# Autodesk Inventor assembly: Pok Mk2
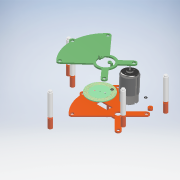
[picture p0: Inventor's stored thumbnail of the model, 180x180]
Saved by Autodesk Inventor 2018.2 (Build 222227000, 227)
## iProperties
Created: 2018-02-07
Part Number: Pok Mk2
Document SubType Name: Assembly
Designer: Moochster
Author: Moochster
## Documents named in this file (10)
- C:\Users\Moochster\OneDrive\Documents\2018 UBC\ELEC 391\Controller\CAD\Pok Mk2.iam
- C:\Users\Moochster\OneDrive\Documents\2018 UBC\ELEC 391\Controller\CAD\JD5B-2655W-R.ipt
- C:\Users\Moochster\OneDrive\Documents\2018 UBC\ELEC 391\Controller\CAD\Encoder Wheel (G16).ipt
- C:\Users\Moochster\OneDrive\Documents\2018 UBC\ELEC 391\Controller\CAD\Pok Yaw Motor Face Mount.ipt
- C:\Users\Moochster\OneDrive\Documents\2018 UBC\ELEC 391\Controller\CAD\Pok Washer I2mmO5mm.ipt
- C:\Users\Moochster\OneDrive\Documents\2018 UBC\ELEC 391\Controller\CAD\Shaft Washer.ipt
- C:\Users\Moochster\OneDrive\Documents\2018 UBC\ELEC 391\Controller\CAD\GP1A52HRJ00F (Large slot detector).ipt
- C:\Users\Moochster\OneDrive\Documents\2018 UBC\ELEC 391\Controller\CAD\Pok X-Carriage Bottom Support.ipt
- C:\Users\Moochster\OneDrive\Documents\2018 UBC\ELEC 391\Controller\CAD\Pok X-Carriage Top Support.ipt
- C:\Users\Moochster\OneDrive\Documents\2018 UBC\ELEC 391\Controller\CAD\Pok Y-Carriage.ipt
## Components (19 placed, 9 different names)
1. JD5B-2655W-R:1
2. Encoder Wheel (G16):1
3. Pok Yaw Motor Face Mount:1
4. Pok Washer I2mmO5mm:1
5. Pok Washer I2mmO5mm:2
6. Shaft Washer:1
7. GP1A52HRJ00F (Large slot detector):1 — Mate:12, Flush:1, Flush:2
8. GP1A52HRJ00F (Large slot detector):2 — Mate:12, Flush:1, Flush:2, Angle:2
9. Pok X-Carriage Bottom Support:1 — Insert:2
10. Pok X-Carriage Bottom Support:2 — Mate:28, Insert:3
11. Pok X-Carriage Bottom Support:3 — Insert:10
12. Pok X-Carriage Bottom Support:4 — Insert:9
13. Pok X-Carriage Bottom Support:5 — Insert:1
14. Pok X-Carriage Top Support:1 — Insert:2
15. Pok X-Carriage Top Support:2 — Insert:1
16. Pok X-Carriage Top Support:3 — Insert:3
17. Pok X-Carriage Top Support:4 — Insert:10
18. Pok X-Carriage Top Support:5 — Insert:9
19. Pok Y-Carriage:1
## Relationships (10: Insert 5, Mate 2, Flush 2, Angle 1)
- Mate:12: GP1A52HRJ00F (Large slot detector):1 ↔ GP1A52HRJ00F (Large slot detector):2
- Flush:1: GP1A52HRJ00F (Large slot detector):1 ↔ GP1A52HRJ00F (Large slot detector):2
- Flush:2: GP1A52HRJ00F (Large slot detector):1 ↔ GP1A52HRJ00F (Large slot detector):2
- Angle:2 (0 deg): GP1A52HRJ00F (Large slot detector):2
- Mate:28: Pok X-Carriage Bottom Support:2
- Insert:1 (0.1 mm): Pok X-Carriage Bottom Support:5 ↔ Pok X-Carriage Top Support:2
- Insert:2 (0.1 mm): Pok X-Carriage Bottom Support:1 ↔ Pok X-Carriage Top Support:1
- Insert:3 (0.1 mm): Pok X-Carriage Bottom Support:2 ↔ Pok X-Carriage Top Support:3
- Insert:9 (0.1 mm): Pok X-Carriage Bottom Support:4 ↔ Pok X-Carriage Top Support:5
- Insert:10 (0.1 mm): Pok X-Carriage Bottom Support:3 ↔ Pok X-Carriage Top Support:4
